# Autodesk Inventor assembly: elric20-2A
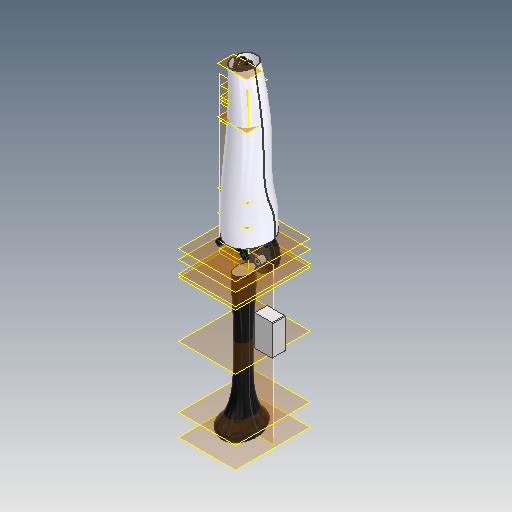
[picture p0: Inventor's stored thumbnail of the model, 512x512]
Saved by Autodesk Inventor 2020.2 (Build 242310000, 310)
## iProperties
Created: 2020-04-12
Part Number: elric20-2A
Document SubType Name: Assembly
Designer: Bardo91
Author: Bardo91
## Documents named in this file (11)
- D:\programming\elric\hardware\2. arm\elric20-02A.iam
- D:\programming\elric\hardware\2. arm\wrist.ipt
- D:\programming\elric\hardware\2. arm\forearm.ipt
- D:\programming\elric\hardware\2. arm\case\arm_case_1.ipt
- D:\programming\elric\hardware\2. arm\case\arm_case_2.ipt
- D:\programming\elric\hardware\2. arm\motor_dc_20d_12v.ipt
- D:\programming\elric\hardware\2. arm\elbow_gear_ext.ipt
- D:\programming\elric\hardware\2. arm\elbow_gear_int_1.ipt
- D:\programming\elric\hardware\2. arm\elbow_gear_int_2.ipt
- D:\programming\elric\hardware\2. arm\arm.ipt
- D:\programming\elric\hardware\2. arm\motor_dc_12v_90d.ipt
## Components (12 placed, 9 different names)
1. wrist:1 — Mate:3, Mate:4
2. forearm:1 — Mate:1, Mate:2, Mate:3, Mate:4
3. motor_dc_20d_12v:1 — Mate:1, Mate:2
4. Spur Gear1:1
5. Spur Gear2:1
6. Spur Gear2:2
7. Spur Gear2:3
8. Spur Gear2:4
9. arm:1
10. motor_dc_12v_90d:1
11. arm_case_1:1
12. arm_case_2:1
## Relationships (18: Mate 11, Flush 7)
- [Flush]: arm_case_1:1 ↔ arm_case_2:1
- [Flush]: arm_case_1:1 ↔ arm_case_2:1
- [Flush]: arm_case_1:1 ↔ arm_case_2:1
- Mate:1: forearm:1 ↔ motor_dc_20d_12v:1
- Mate:2: forearm:1 ↔ motor_dc_20d_12v:1
- Mate:3: wrist:1 ↔ forearm:1
- Mate:4 (0.5 mm): wrist:1 ↔ forearm:1
- [Mate]: forearm:1 ↔ Spur Gear1:1
- [Mate]: forearm:1 ↔ Spur Gear1:1
- [Mate]: forearm:1 ↔ Spur Gear1:1
- [Mate]: Spur Gear2:2 ↔ arm:1
- [Flush]: Spur Gear2:3 ↔ Spur Gear2:4
- [Flush]: Spur Gear2:1 ↔ Spur Gear2:4
- [Flush]: Spur Gear2:2 ↔ Spur Gear2:4
- [Mate]: Spur Gear1:1 ↔ Spur Gear2:4
- [Flush]: Spur Gear1:1 ↔ Spur Gear2:4
- [Mate]: Spur Gear2:1 ↔ arm:1
- [Mate]: Spur Gear2:3 ↔ arm:1
## Named parameters: d28_d7 = 0 mm, d29_d8 = 0 mm, d30_d9 = 0 mm
